# Autodesk Inventor assembly: roller cage
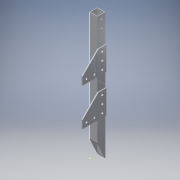
[picture p0: Inventor's stored thumbnail of the model, 180x180]
Saved by Autodesk Inventor 2016 (Build 200138000, 138)
## iProperties
Created: 2016-02-02
Part Number: roller cage
Document SubType Name: Assembly
Designer: gus
Mass: 261.186 g
Surface Area: 977.44 cm^2
Volume: 96.7354 cm^3
Density: 2.7 g/cm^3
Author: gus
## Documents named in this file (4)
- \\Mac\Home\Desktop\1510-stronghold-CAD-master\roller cage\roller cage.iam
- \\Mac\Home\Desktop\1510-stronghold-CAD-master\roller cage\top.ipt
- \\Mac\Home\Desktop\1510-stronghold-CAD-master\roller cage\gusset plate.ipt
- \\Mac\Home\Desktop\1510-stronghold-CAD-master\roller cage\robot.iam
## Components (4 placed, 3 different names)
1. top:1 — Mate:3, Mate:7, Mate:8, Mate:9, Mate:10, Mate:11
2. gusset plate:2 — Mate:3, Mate:7, Mate:8
3. robot:1 [sub-assembly]
4. gusset plate:3 — Mate:9, Mate:10, Mate:11
## Relationships (6: Mate 6)
- Mate:3: top:1 ↔ gusset plate:2
- Mate:7: top:1 ↔ gusset plate:2
- Mate:8: top:1 ↔ gusset plate:2
- Mate:9: top:1 ↔ gusset plate:3
- Mate:10: top:1 ↔ gusset plate:3
- Mate:11: top:1 ↔ gusset plate:3
